# Autodesk Inventor assembly: base plate
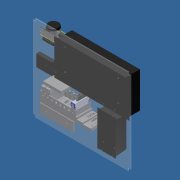
[picture p0: Inventor's stored thumbnail of the model, 180x180]
Saved by Autodesk Inventor 2012 (Build 160160000, 160)
## iProperties
Created: 2012-05-12
Part Number: base plate
Document SubType Name: Assembly
Designer: esv
Mass: 10089.4 g
Surface Area: 12680.2 cm^2
Volume: 8294.97 cm^3
Density: 1.21633 g/cm^3
Author: esv
## Documents named in this file (10)
- C:\Users\Ed\Documents\masters\CAD\base plate.iam
- C:\Users\Ed\Documents\masters\CAD\cRIO\Inventor\cRIO with Modules.iam
- C:\Users\Ed\Documents\masters\CAD\Cap\Cap.ipt
- C:\Users\Ed\Documents\masters\CAD\Frame\base plate.ipt
- C:\Users\Ed\Documents\masters\CAD\cRIO\cRIO Breakout Keepout.ipt
- C:\Users\Ed\Documents\masters\CAD\13.8V Supply\supply-13.8.ipt
- C:\Users\Ed\Documents\masters\CAD\Sabertooth\sabertooth keepout.ipt
- C:\Users\Ed\Documents\masters\CAD\cRIO\cRIO bracket.ipt
- C:\Users\Ed\Documents\masters\CAD\Relay\relay.ipt
- C:\Users\Ed\Documents\masters\CAD\Inverter\2kW inverter.ipt
## Components (9 placed, 9 different names)
1. cRIO with Modules:1 [sub-assembly] — Mate:1, Flush:1, Flush:2, Insert:6, Insert:7
2. Cap:1 — Tangent:1, Flush:3, Tangent:2
3. base plate:1 — Insert:8, Insert:9, Insert:10, Angle:2, Mate:2, Flush:4, Flush:5, Flush:6, Mate:3, Mate:4, Flush:7, Flush:9
4. cRIO Breakout Keepout:1 — Mate:1, Flush:1, Flush:2
5. supply-13.8:1 — Flush:6, Mate:3, Flush:9
6. sabertooth keepout:1 — Mate:4, Flush:7, Flush:8
7. cRIO bracket:1 — Insert:6, Insert:7, Insert:8, Insert:9, Tangent:1, Flush:3, Tangent:2
8. relay:1 — Insert:10, Angle:2
9. 2kW inverter:1 — Mate:2, Flush:4, Flush:5, Flush:8
## Relationships (21: Flush 9, Insert 5, Mate 4, Tangent 2, Angle 1)
- Mate:1: cRIO with Modules:1 ↔ cRIO Breakout Keepout:1
- Flush:1: cRIO with Modules:1 ↔ cRIO Breakout Keepout:1
- Flush:2: cRIO with Modules:1 ↔ cRIO Breakout Keepout:1
- Insert:6: cRIO with Modules:1 ↔ cRIO bracket:1
- Insert:7: cRIO with Modules:1 ↔ cRIO bracket:1
- Insert:8: base plate:1 ↔ cRIO bracket:1
- Insert:9: base plate:1 ↔ cRIO bracket:1
- Tangent:1: Cap:1 ↔ cRIO bracket:1
- Flush:3 (50.8 mm): Cap:1 ↔ cRIO bracket:1
- Tangent:2: Cap:1 ↔ cRIO bracket:1
- Insert:10: base plate:1 ↔ relay:1
- Angle:2 (0 deg): base plate:1 ↔ relay:1
- Mate:2: base plate:1 ↔ 2kW inverter:1
- Flush:4 (-25.4 mm): base plate:1 ↔ 2kW inverter:1
- Flush:5 (19.05 mm): base plate:1 ↔ 2kW inverter:1
- Flush:6 (-76.2 mm): base plate:1 ↔ supply-13.8:1
- Mate:3: base plate:1 ↔ supply-13.8:1
- Mate:4: base plate:1 ↔ sabertooth keepout:1
- Flush:7: base plate:1 ↔ sabertooth keepout:1
- Flush:8: sabertooth keepout:1 ↔ 2kW inverter:1
- Flush:9 (-6.35 mm): base plate:1 ↔ supply-13.8:1
